# Autodesk Inventor assembly: ArduinoMegaWithCase
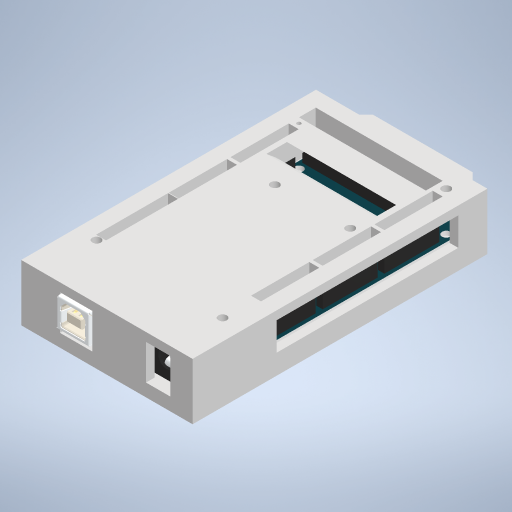
[picture p0: Inventor's stored thumbnail of the model, 512x512]
Saved by Autodesk Inventor 2024 (Build 280153000, 153)
## iProperties
Created: 2023-07-08
Part Number: ArduinoMegaWithCase
Document SubType Name: Assembly
Designer: 18179
Author: 18179
## Documents named in this file (4)
- C:\Users\18179\Desktop\TuppyMkIV\ArduinoMegaWithCase.iam
- C:\Users\18179\Desktop\TuppyMkIV\ArduinoMegaCaseBottom.ipt
- C:\Users\18179\Downloads\arduino-mega-2560-9.snapshot.4\arduino_MEGA2560\arduino_MEGA2560.iam
- C:\Users\18179\Desktop\TuppyMkIV\ArduinoMegaCaseTop.ipt
## Components (3 placed, 3 different names)
1. arduino_MEGA2560:1 [sub-assembly] — Mate:1, Mate:2, Mate:3
2. ArduinoMegaCaseBottom:1 — Mate:1, Mate:2, Mate:3, Mate:4, Flush:1, Flush:2
3. ArduinoMegaCaseTop:1 — Mate:4, Flush:1, Flush:2
## Relationships (6: Mate 4, Flush 2)
- Mate:1: arduino_MEGA2560:1 ↔ ArduinoMegaCaseBottom:1
- Mate:2: arduino_MEGA2560:1 ↔ ArduinoMegaCaseBottom:1
- Mate:3: arduino_MEGA2560:1 ↔ ArduinoMegaCaseBottom:1
- Mate:4: ArduinoMegaCaseBottom:1 ↔ ArduinoMegaCaseTop:1
- Flush:1: ArduinoMegaCaseBottom:1 ↔ ArduinoMegaCaseTop:1
- Flush:2: ArduinoMegaCaseBottom:1 ↔ ArduinoMegaCaseTop:1
